# Autodesk Inventor assembly: 回路ボックス1
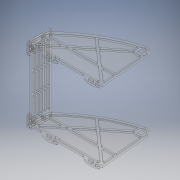
[picture p0: Inventor's stored thumbnail of the model, 180x180]
Saved by Autodesk Inventor 2020 (Build 240168000, 168)
## iProperties
Created: 2019-09-10
Part Number: 回路ボックス1
Document SubType Name: Assembly
Designer: 雪村
Mass: 30.5146 g
Surface Area: 406.954 cm^2
Volume: 25.4288 cm^3
Density: 1.2 g/cm^3
Author: 雪村
## Documents named in this file (5)
- C:\Users\white\Documents\SRDC\SRDC\Inventor_2017\2018年機体\2020年4年機体\回路ボックス1.iam
- C:\Users\white\Documents\SRDC\SRDC\Inventor_2017\2018年機体\2020年4年機体\回路ボックス1.1.ipt
- C:\Users\white\Documents\SRDC\SRDC\Inventor_2017\2018年機体\2020年4年機体\回路ボックス1.2.ipt
- C:\Users\white\Documents\SRDC\SRDC\Inventor_2017\2018年機体\2020年4年機体\回路ボックス1.1_MIR.ipt
- C:\Users\white\Documents\SRDC\SRDC\Inventor_2017\2018年機体\パーツ\アームユニット底板締結パーツ3t用(4).ipt
## Components (5 placed, 4 different names)
1. 回路ボックス1.1:1 — メイト:1, メイト:3, メイト:4
2. 回路ボックス1.2:1 — メイト:1, メイト:2, メイト:3, メイト:4, メイト:5, メイト:6, メイト:7, メイト:8, メイト:9, メイト:10, メイト:11, メイト:12
3. 回路ボックス1.1_MIR:1 — メイト:2, メイト:5, メイト:6
4. アームユニット底板締結パーツ3t用(4):1 — メイト:8, メイト:9, メイト:12
5. アームユニット底板締結パーツ3t用(4):2 — メイト:7, メイト:10, メイト:11
## Relationships (12: Mate 12)
- メイト:1 [Mate]: 回路ボックス1.1:1 ↔ 回路ボックス1.2:1
- メイト:2 [Mate]: 回路ボックス1.2:1 ↔ 回路ボックス1.1_MIR:1
- メイト:3 [Mate]: 回路ボックス1.1:1 ↔ 回路ボックス1.2:1
- メイト:4 [Mate]: 回路ボックス1.1:1 ↔ 回路ボックス1.2:1
- メイト:5 [Mate]: 回路ボックス1.2:1 ↔ 回路ボックス1.1_MIR:1
- メイト:6 [Mate]: 回路ボックス1.2:1 ↔ 回路ボックス1.1_MIR:1
- メイト:7 [Mate]: 回路ボックス1.2:1 ↔ アームユニット底板締結パーツ3t用(4):2
- メイト:8 [Mate]: 回路ボックス1.2:1 ↔ アームユニット底板締結パーツ3t用(4):1
- メイト:9 [Mate]: 回路ボックス1.2:1 ↔ アームユニット底板締結パーツ3t用(4):1
- メイト:10 [Mate]: 回路ボックス1.2:1 ↔ アームユニット底板締結パーツ3t用(4):2
- メイト:11 [Mate]: 回路ボックス1.2:1 ↔ アームユニット底板締結パーツ3t用(4):2
- メイト:12 [Mate]: 回路ボックス1.2:1 ↔ アームユニット底板締結パーツ3t用(4):1
